# Autodesk Inventor assembly: wheel_mechanism
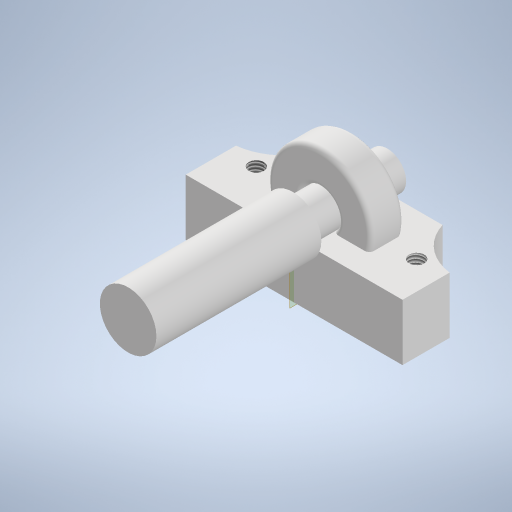
[picture p0: Inventor's stored thumbnail of the model, 512x512]
Saved by Autodesk Inventor 2024 (Build 280153000, 153)
## iProperties
Created: 2023-08-23
Part Number: wheel_mechanism
Document SubType Name: Assembly
Designer: Pintu
Author: Pintu
## Documents named in this file (4)
- D:\CMC\my_inventor\ArmBo_v2\HOLDERS\wheel_mechanism.iam
- D:\CMC\my_inventor\ArmBo_v2\HOLDERS\bearing_wheel_holder.ipt
- D:\CMC\my_inventor\ArmBo_v2\HOLDERS\bearing.ipt
- D:\CMC\my_inventor\ArmBo_v2\HOLDERS\shaft_optical_enc.ipt
## Components (3 placed, 3 different names)
1. bearing_wheel_holder:1
2. bearing:1 — Mate:1
3. shaft_optical_enc:1 — Mate:1
## Relationships (1: Mate 1)
- Mate:1: bearing:1 ↔ shaft_optical_enc:1
